# Autodesk Inventor assembly: fan
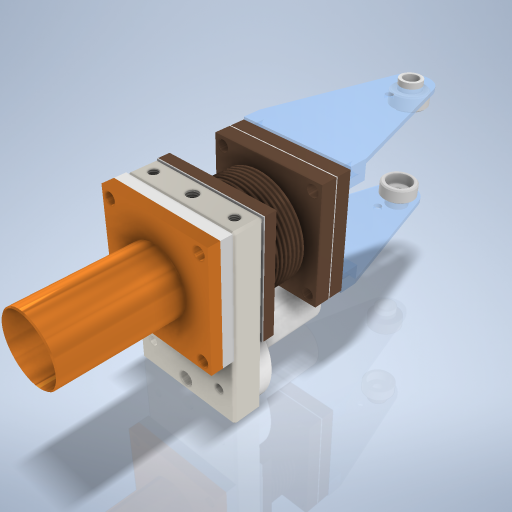
[picture p0: Inventor's stored thumbnail of the model, 512x512]
Saved by Autodesk Inventor 2024.2 (Build 282272000, 272)
## iProperties
Created: 2024-05-16
Part Number: fan
Document SubType Name: Assembly
Designer: Fabri
Author: Fabri
## Documents named in this file (11)
- C:\Users\Fabri\Documents\Inventor\Stirlingfan\fan.iam
- C:\Users\Fabri\Documents\Inventor\Stirlingfan\cylinder.ipt
- C:\Users\Fabri\Documents\Inventor\Stirlingfan\05.ipt
- C:\Users\Fabri\Documents\Inventor\Stirlingfan\sheet_cylinder.ipt
- C:\Users\Fabri\Documents\Inventor\Stirlingfan\8.ipt
- C:\Users\Fabri\Documents\Inventor\Stirlingfan\cylinder_lid.ipt
- C:\Users\Fabri\Documents\Inventor\Stirlingfan\07.ipt
- C:\Users\Fabri\Documents\Inventor\Stirlingfan\01.ipt
- C:\Users\Fabri\Documents\Inventor\Stirlingfan\11.ipt
- C:\Users\Fabri\Documents\Inventor\Stirlingfan\thickshield_cylinder.ipt
- C:\Users\Fabri\Documents\Inventor\Stirlingfan\candle_cylinder.ipt
## Components (13 placed, 10 different names)
1. cylinder:1 — Passend:17, Einfügen:26, Passend:18, Einfügen:27, Passend:19
2. 05:1 — Passend:3, Einfügen:6, Passend:10, Passend:11, Einfügen:19
3. 05:2 — Passend:4, Einfügen:5, Einfügen:20
4. sheet_cylinder:2 — Passend:18, Einfügen:27, Einfügen:28
5. sheet_cylinder:3 — Passend:13, Passend:14, Einfügen:22, Einfügen:26
6. 8:1 — Passend:4, Einfügen:5
7. 8:2 — Passend:3, Einfügen:6
8. 07:1 — Passend:9, Einfügen:17
9. 01:1 — Passend:6, Einfügen:12, Passend:13, Passend:14, Einfügen:22, Passend:16, Einfügen:25, Passend:17
10. 11:1 — Passend:6, Einfügen:12
11. thickshield_cylinder:1 — Passend:15, Einfügen:24, Passend:16, Einfügen:25
12. candle_cylinder:1 — Passend:15, Einfügen:24
13. cylinder_lid:1 — Passend:9, Einfügen:17, Passend:10, Passend:11, Einfügen:19, Einfügen:20, Passend:19, Einfügen:28
## Relationships (25: Mate 13, Insert 12)
- Passend:3 [Mate]: 05:1 ↔ 8:2
- Passend:4 [Mate]: 05:2 ↔ 8:1
- Einfügen:5 [Insert]: 05:2 ↔ 8:1
- Einfügen:6 [Insert]: 05:1 ↔ 8:2
- Passend:6 [Mate]: 01:1 ↔ 11:1
- Einfügen:12 [Insert]: 01:1 ↔ 11:1
- Passend:9 [Mate]: 07:1 ↔ cylinder_lid:1
- Einfügen:17 [Insert]: 07:1 ↔ cylinder_lid:1
- Passend:10 [Mate]: 05:1 ↔ cylinder_lid:1
- Passend:11 [Mate]: 05:1 ↔ cylinder_lid:1
- Einfügen:19 [Insert]: 05:1 ↔ cylinder_lid:1
- Einfügen:20 [Insert]: 05:2 ↔ cylinder_lid:1
- Passend:13 [Mate]: sheet_cylinder:3 ↔ 01:1
- Passend:14 [Mate]: sheet_cylinder:3 ↔ 01:1
- Einfügen:22 [Insert]: sheet_cylinder:3 ↔ 01:1
- Passend:15 [Mate]: thickshield_cylinder:1 ↔ candle_cylinder:1
- Einfügen:24 [Insert]: thickshield_cylinder:1 ↔ candle_cylinder:1
- Passend:16 [Mate]: 01:1 ↔ thickshield_cylinder:1
- Einfügen:25 [Insert]: 01:1 ↔ thickshield_cylinder:1
- Passend:17 [Mate]: cylinder:1 ↔ 01:1
- Einfügen:26 [Insert]: cylinder:1 ↔ sheet_cylinder:3
- Passend:18 [Mate]: cylinder:1 ↔ sheet_cylinder:2
- Einfügen:27 [Insert]: cylinder:1 ↔ sheet_cylinder:2
- Passend:19 [Mate]: cylinder:1 ↔ cylinder_lid:1
- Einfügen:28 [Insert]: sheet_cylinder:2 ↔ cylinder_lid:1
